# Autodesk Inventor assembly: YAxisIdlerLeft
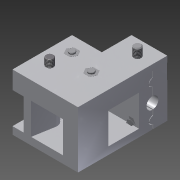
[picture p0: Inventor's stored thumbnail of the model, 180x180]
Saved by Autodesk Inventor 2015 (Build 190159000, 159)
## iProperties
Created: 2014-08-09
Part Number: YAxisIdlerLeft
Document SubType Name: Assembly
Designer: Jack
Author: Jack
## Documents named in this file (11)
- C:\Users\Jack\ownCloud\Projects\CoreXY\InventorModel\Old\YAxis\YAxisIdler\YAxisIdlerLeft.old.iam
- C:\Users\Jack\ownCloud\Projects\CoreXY\InventorModel\Old\YAxis\YAxisIdler\YAxisIdlerBlock.old.ipt
- C:\Users\Jack\ownCloud\Projects\CoreXY\InventorModel\Old\YAxis\YAxisIdler\YAxisIdlerCap.old.ipt
- C:\Users\Jack\ownCloud\Projects\CoreXY\InventorModel\Hardware\Bolts\SHCS\SHCS4\SHCS4x35.ipt
- C:\Users\Jack\ownCloud\Projects\CoreXY\InventorModel\Hardware\Nuts\Nut4.ipt
- C:\Users\Jack\ownCloud\Projects\CoreXY\InventorModel\Hardware\Bolts\SHCS\SHCS4\SHCS4x15.ipt
- C:\Users\Jack\ownCloud\Projects\CoreXY\InventorModel\Hardware\Bolts\SHCS\SHCS5\SHCS5x10.ipt
- C:\Users\Jack\ownCloud\Projects\CoreXY\InventorModel\Hardware\Bolts\FHS\FHS5\5x10FHS.ipt
- C:\Users\Jack\ownCloud\Projects\CoreXY\InventorModel\Hardware\Bearing\BearingRadialBall\BearingRadialBallF624zz.ipt
- C:\Users\Jack\ownCloud\Projects\CoreXY\InventorModel\Hardware\Wahsers\M4Washer.ipt
- C:\Users\Jack\ownCloud\Projects\CoreXY\InventorModel\Old\YAxis\YAxisIdler\YAxisIdlerBearingSpacer.old.ipt
## Components (24 placed, 10 different names)
1. YAxisIdlerBlock.old:1 — Mate:1, Flush:2, Mate:2, Mate:3, Flush:3, Mate:4, Mate:5, Mate:6, Mate:7, Mate:10, Mate:11, Angle:1, Angle:2, Mate:12, Mate:14, Mate:20, Flush:4, Mate:21, Mate:22, Mate:36, Mate:38, Mate:39, Mate:40, Mate:41, Mate:42
2. YAxisIdlerCap.old:1 — Mate:1, Flush:2, Mate:16, Mate:17, Mate:18, Mate:19
3. SHCS4x35:1 — Mate:4, Mate:7, Mate:8, Mate:35, Mate:44
4. SHCS4x35:2 — Mate:5, Mate:6, Mate:9, Mate:37, Mate:45
5. Nut4:1 — Mate:8, Mate:10, Angle:2
6. Nut4:2 — Mate:9, Mate:11, Angle:1
7. Nut4:3 — Mate:14
8. Nut4:4 — Mate:12
9. SHCS4x15:1 — Mate:16, Mate:18
10. SHCS4x15:2 — Mate:17, Mate:19
11. SHCS5x10:1 — Mate:21, Mate:22
12. 5x10FHS:1 — Mate:20, Flush:4
13. BearingRadialBallF624zz:1
14. BearingRadialBallF624zz:2
15. M4Washer:1 — Mate:46
16. M4Washer:2 — Mate:37, Mate:38
17. BearingRadialBallF624zz:3
18. BearingRadialBallF624zz:4
19. M4Washer:3 — Mate:36
20. M4Washer:4 — Mate:35, Mate:43
21. SHCS5x10:2 — Mate:39, Mate:42
22. SHCS5x10:3 — Mate:40, Mate:41
23. YAxisIdlerBearingSpacer.old:1 — Mate:43, Mate:44
24. YAxisIdlerBearingSpacer.old:2 — Mate:45, Mate:46
## Relationships (49: Mate 44, Flush 3, Angle 2)
- Mate:1: YAxisIdlerBlock.old:1 ↔ YAxisIdlerCap.old:1
- Flush:2: YAxisIdlerBlock.old:1 ↔ YAxisIdlerCap.old:1
- Mate:2: YAxisIdlerBlock.old:1
- Mate:3: YAxisIdlerBlock.old:1
- Flush:3: YAxisIdlerBlock.old:1
- Mate:4: YAxisIdlerBlock.old:1 ↔ SHCS4x35:1
- Mate:5: YAxisIdlerBlock.old:1 ↔ SHCS4x35:2
- Mate:6: YAxisIdlerBlock.old:1 ↔ SHCS4x35:2
- Mate:7: YAxisIdlerBlock.old:1 ↔ SHCS4x35:1
- Mate:8: SHCS4x35:1 ↔ Nut4:1
- Mate:9: SHCS4x35:2 ↔ Nut4:2
- Mate:10: YAxisIdlerBlock.old:1 ↔ Nut4:1
- Mate:11: YAxisIdlerBlock.old:1 ↔ Nut4:2
- Angle:1 (0 deg): YAxisIdlerBlock.old:1 ↔ Nut4:2
- Angle:2 (0 deg): YAxisIdlerBlock.old:1 ↔ Nut4:1
- Mate:12: YAxisIdlerBlock.old:1 ↔ Nut4:4
- Mate:14: YAxisIdlerBlock.old:1 ↔ Nut4:3
- Mate:16: YAxisIdlerCap.old:1 ↔ SHCS4x15:1
- Mate:17: YAxisIdlerCap.old:1 ↔ SHCS4x15:2
- Mate:18: YAxisIdlerCap.old:1 ↔ SHCS4x15:1
- Mate:19: YAxisIdlerCap.old:1 ↔ SHCS4x15:2
- Mate:20: YAxisIdlerBlock.old:1 ↔ 5x10FHS:1
- Flush:4: YAxisIdlerBlock.old:1 ↔ 5x10FHS:1
- Mate:21: YAxisIdlerBlock.old:1 ↔ SHCS5x10:1
- Mate:22: YAxisIdlerBlock.old:1 ↔ SHCS5x10:1
- [Mate]: BearingRadialBallF624zz:1 ↔ BearingRadialBallF624zz:2
- [Mate]: BearingRadialBallF624zz:1 ↔ BearingRadialBallF624zz:2
- [Mate]: BearingRadialBallF624zz:1 ↔ M4Washer:1
- [Mate]: BearingRadialBallF624zz:2 ↔ M4Washer:1
- [Mate]: BearingRadialBallF624zz:1 ↔ M4Washer:2
- [Mate]: BearingRadialBallF624zz:1 ↔ M4Washer:2
- [Mate]: BearingRadialBallF624zz:3 ↔ BearingRadialBallF624zz:4
- [Mate]: BearingRadialBallF624zz:3 ↔ BearingRadialBallF624zz:4
- [Mate]: BearingRadialBallF624zz:3 ↔ M4Washer:3
- [Mate]: BearingRadialBallF624zz:4 ↔ M4Washer:3
- [Mate]: BearingRadialBallF624zz:3 ↔ M4Washer:4
- [Mate]: BearingRadialBallF624zz:3 ↔ M4Washer:4
- Mate:35: SHCS4x35:1 ↔ M4Washer:4
- Mate:36: YAxisIdlerBlock.old:1 ↔ M4Washer:3
- Mate:37: SHCS4x35:2 ↔ M4Washer:2
- Mate:38: YAxisIdlerBlock.old:1 ↔ M4Washer:2
- Mate:39: YAxisIdlerBlock.old:1 ↔ SHCS5x10:2
- Mate:40: YAxisIdlerBlock.old:1 ↔ SHCS5x10:3
- Mate:41: YAxisIdlerBlock.old:1 ↔ SHCS5x10:3
- Mate:42: YAxisIdlerBlock.old:1 ↔ SHCS5x10:2
- Mate:43: M4Washer:4 ↔ YAxisIdlerBearingSpacer.old:1
- Mate:44: SHCS4x35:1 ↔ YAxisIdlerBearingSpacer.old:1
- Mate:45: SHCS4x35:2 ↔ YAxisIdlerBearingSpacer.old:2
- Mate:46: M4Washer:1 ↔ YAxisIdlerBearingSpacer.old:2
## Named parameters: d63_d160 = 0 mm, d64_d161 = 0 mm, d65_d162 = 0 mm, d66_d163 = 0 mm, d67_d158 = 0 mm, d68_d159 = 0 mm
